# Autodesk Inventor assembly: Sorting Mechanism Assembly
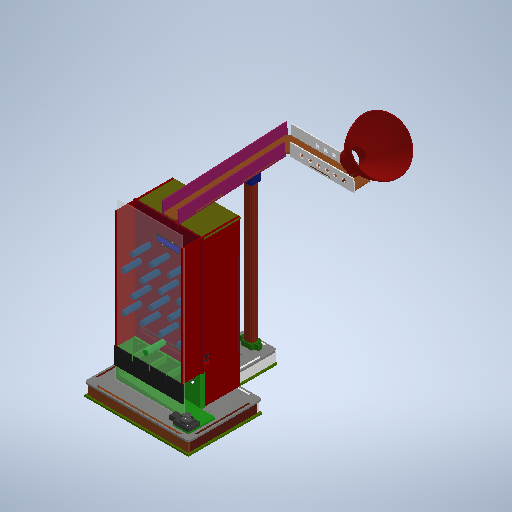
[picture p0: Inventor's stored thumbnail of the model, 512x512]
Saved by Autodesk Inventor 2025.4 (Build 294407000, 407)
## iProperties
Created: 2026-04-05
Part Number: Sorting Mechanism Assembly
Document SubType Name: Assembly
Designer: lenovo
Author: lenovo
## Documents named in this file (39)
- F:\ASU Engineering\Year.2 ( 25-26 )\Spring\Basics Of Mechatronics\Project\Mechanisms\Sorting Mechanism\Sorting Mechanism Assembly.iam
- F:\ASU Engineering\Year.2 ( 25-26 )\Spring\Basics Of Mechatronics\Project\Mechanisms\Sorting Mechanism\Base.ipt
- F:\ASU Engineering\Year.2 ( 25-26 )\Spring\Basics Of Mechatronics\Project\Mechanisms\Sorting Mechanism\Random Plate  ( Laser Cut ).ipt
- F:\ASU Engineering\Year.2 ( 25-26 )\Spring\Basics Of Mechatronics\Project\Mechanisms\Sorting Mechanism\Randomization Stick.ipt
- F:\ASU Engineering\Year.2 ( 25-26 )\Spring\Basics Of Mechatronics\Project\Mechanisms\Sorting Mechanism\Finishing Sheets .1  ( Right ).ipt
- F:\ASU Engineering\Year.2 ( 25-26 )\Spring\Basics Of Mechatronics\Project\Mechanisms\Sorting Mechanism\Rack ( Female Fixation ).ipt
- F:\ASU Engineering\Year.2 ( 25-26 )\Spring\Basics Of Mechatronics\Project\Mechanisms\Sorting Mechanism\Rack ( Male Fixation.ipt
- F:\ASU Engineering\Year.2 ( 25-26 )\Spring\Basics Of Mechatronics\Project\Mechanisms\Sorting Mechanism\Sorting Mechanism Base Fixation.ipt
- F:\ASU Engineering\Year.2 ( 25-26 )\Spring\Basics Of Mechatronics\Project\Mechanisms\Sorting Mechanism\Finishing Sheets .2  ( Upper ).ipt
- F:\ASU Engineering\Year.2 ( 25-26 )\Spring\Basics Of Mechatronics\Project\Mechanisms\Sorting Mechanism\Finishing Sheets .3  ( Back ).ipt
- F:\ASU Engineering\Year.2 ( 25-26 )\Spring\Basics Of Mechatronics\Project\Mechanisms\Sorting Mechanism\Finishing Sheets .4 ( Front )  Acrylic.ipt
- F:\ASU Engineering\Year.2 ( 25-26 )\Spring\Basics Of Mechatronics\Project\Mechanisms\Sorting Mechanism\Finishing Sheets .5 ( Buttom ).ipt
- F:\ASU Engineering\Year.2 ( 25-26 )\Spring\Basics Of Mechatronics\Project\Mechanisms\Sorting Mechanism\Joystick Shield.ipt
- F:\ASU Engineering\Year.2 ( 25-26 )\Spring\Basics Of Mechatronics\Project\Mechanisms\Sorting Mechanism\Base Leg V1.ipt
- F:\ASU Engineering\Year.2 ( 25-26 )\Spring\Basics Of Mechatronics\Project\Mechanisms\Sorting Mechanism\Base Leg V2.ipt
- F:\ASU Engineering\Year.2 ( 25-26 )\Spring\Basics Of Mechatronics\Project\Mechanisms\Sorting Mechanism\Movable Stick.ipt
- F:\ASU Engineering\Year.2 ( 25-26 )\Spring\Basics Of Mechatronics\Project\Mechanisms\Sorting Mechanism\Lower Path Fixation.ipt
- F:\ASU Engineering\Year.2 ( 25-26 )\Spring\Basics Of Mechatronics\Project\Mechanisms\Sorting Mechanism\Path Holder.ipt
- F:\ASU Engineering\Year.2 ( 25-26 )\Spring\Basics Of Mechatronics\Project\Mechanisms\Sorting Mechanism\Upper Path Fixation.ipt
- F:\ASU Engineering\Year.2 ( 25-26 )\Spring\Basics Of Mechatronics\Project\Mechanisms\Sorting Mechanism\Path.ipt
- F:\ASU Engineering\Year.2 ( 25-26 )\Spring\Basics Of Mechatronics\Project\Mechanisms\Sorting Mechanism\Path Side Wall.ipt
- F:\ASU Engineering\Year.2 ( 25-26 )\Spring\Basics Of Mechatronics\Project\Mechanisms\Sorting Mechanism\Path Back End.ipt
- F:\ASU Engineering\Year.2 ( 25-26 )\Spring\Basics Of Mechatronics\Project\Mechanisms\Sorting Mechanism\Cone FV.ipt
- F:\ASU Engineering\Year.2 ( 25-26 )\Spring\Basics Of Mechatronics\Project\Mechanisms\Sorting Mechanism\Path Base Fixation .1.ipt
- F:\ASU Engineering\Year.2 ( 25-26 )\Spring\Basics Of Mechatronics\Project\Mechanisms\Sorting Mechanism\Path Base Fixation .2.ipt
- F:\ASU Engineering\Year.2 ( 25-26 )\Spring\Basics Of Mechatronics\Project\Mechanisms\Sorting Mechanism\Sensors Shield.ipt
- F:\ASU Engineering\Year.2 ( 25-26 )\Spring\Basics Of Mechatronics\Project\Mechanisms\Sorting Mechanism\DC Gear Motor Single Shaft\DC Gear Motor Single Shaft\DC Gear Motor Single Shaft.ipt
- F:\ASU Engineering\Year.2 ( 25-26 )\Spring\Basics Of Mechatronics\Project\Mechanisms\Sorting Mechanism\IR Sensor\IR Sensor\IR Sensor.ipt
- F:\ASU Engineering\Year.2 ( 25-26 )\Spring\Basics Of Mechatronics\Project\Mechanisms\Sorting Mechanism\Limit_Switch\Limit_Switch\Limit_Switch.ipt
- F:\ASU Engineering\Year.2 ( 25-26 )\Spring\Basics Of Mechatronics\Project\Mechanisms\Sorting Mechanism\Joystick\Joystick\Joystick.ipt
- F:\ASU Engineering\Year.2 ( 25-26 )\Spring\Basics Of Mechatronics\Project\Mechanisms\Sorting Mechanism\Base Leg V2 Slotted.ipt
- F:\ASU Engineering\Year.2 ( 25-26 )\Spring\Basics Of Mechatronics\Project\Mechanisms\Sorting Mechanism\DC Motor Fixing Wall.ipt
- F:\ASU Engineering\Year.2 ( 25-26 )\Spring\Basics Of Mechatronics\Project\Mechanisms\Sorting Mechanism\Geared Motor Transmission.ipt
- F:\ASU Engineering\Year.2 ( 25-26 )\Spring\Basics Of Mechatronics\Project\Mechanisms\Sorting Mechanism\Pinion Gear FV.ipt
- F:\ASU Engineering\Year.2 ( 25-26 )\Spring\Basics Of Mechatronics\Project\Mechanisms\Sorting Mechanism\Path Plate Connector.ipt
- F:\ASU Engineering\Year.2 ( 25-26 )\Spring\Basics Of Mechatronics\Project\Mechanisms\Sorting Mechanism\LCD-I2C_16X2\LCD-I2C_16X2\LCD-I2C_16X2.iam
- F:\ASU Engineering\Year.2 ( 25-26 )\Spring\Basics Of Mechatronics\Project\Mechanisms\Sorting Mechanism\Extension .1.ipt
- F:\ASU Engineering\Year.2 ( 25-26 )\Spring\Basics Of Mechatronics\Project\Mechanisms\Sorting Mechanism\Extension.2.ipt
- F:\ASU Engineering\Year.2 ( 25-26 )\Spring\Basics Of Mechatronics\Project\Mechanisms\Sorting Mechanism\Extension .3.ipt
## Components (63 placed, 38 different names)
1. Base:1 — Mate:1, Mate:3, Flush:1, Mate:34, Mate:37, Mate:48, Mate:49, Mate:50, Mate:62, Mate:63, Mate:64, Mate:127, Mate:128, Mate:129, Mate:130, Mate:131, Mate:132, Mate:133, Mate:134, Mate:135, Mate:136, Mate:137, Mate:138, Mate:139, Mate:140, Mate:147, Mate:153, Mate:167, Mate:168, Mate:169
2. Random Plate  ( Laser Cut ):1 — Mate:1, Mate:3, Flush:1, Mate:4, Mate:5, Mate:6, Mate:7, Mate:8, Mate:9, Mate:10, Mate:11, Mate:12, Mate:13, Mate:14, Mate:15, Mate:16, Mate:17, Mate:18, Mate:19, Mate:20, Mate:21, Mate:22, Mate:23, Mate:24, Mate:25, Mate:26, Mate:27, Mate:28, Mate:29, Mate:30, Mate:31, Mate:32, Mate:33, Mate:35, Mate:36, Mate:38, Mate:39, Mate:40, Mate:51, Mate:59, Mate:79, Mate:80, Mate:124, Mate:175, Mate:177, Mate:178, Mate:179
3. Randomization Stick:1 — Mate:4, Mate:18
4. Randomization Stick:2 — Mate:8, Mate:20
5. Randomization Stick:3 — Mate:5, Mate:19
6. Randomization Stick:4 — Mate:7, Mate:27
7. Randomization Stick:5 — Mate:6, Mate:28
8. Randomization Stick:6 — Mate:9, Mate:30
9. Randomization Stick:7 — Mate:10, Mate:29
10. Randomization Stick:8 — Mate:11, Mate:21
11. Randomization Stick:9 — Mate:12, Mate:22
12. Randomization Stick:10 — Mate:14, Mate:31
13. Randomization Stick:11 — Mate:13, Mate:23
14. Randomization Stick:12 — Mate:16, Mate:25
15. Randomization Stick:13 — Mate:17, Mate:26
16. Randomization Stick:14 — Mate:15, Mate:24
17. Finishing Sheets .1  ( Right ):1 — Mate:32, Mate:33, Mate:34, Mate:80, Mate:126
18. Finishing Sheets .1  ( Right ):2 — Mate:35, Mate:36, Mate:37, Mate:52, Mate:53, Mate:55, Mate:56, Mate:60, Mate:61, Mate:79
19. Rack ( Female Fixation ):1 — Mate:38, Mate:39, Mate:40, Mate:41, Mate:42, Mate:155, Mate:156, Mate:157, Mate:158, Mate:159, Mate:160
20. Rack ( Male Fixation:1 — Mate:41, Mate:42, Mate:81, Mate:82, Rotation/Translation:1
21. Sorting Mechanism Base Fixation:1 — Mate:48, Mate:49, Mate:50, Mate:65, Mate:66, Mate:68, Mate:71, Mate:72, Mate:73, Mate:74, Mate:75, Mate:76, Mate:77, Flush:59, Mate:96, Mate:97, Mate:98, Mate:113, Mate:114, Mate:115, Mate:116, Mate:117, Mate:118, Mate:120, Mate:121, Mate:164, Mate:165, Mate:166
22. Finishing Sheets .2  ( Upper ):1 — Mate:59, Mate:60, Mate:61
23. Finishing Sheets .3  ( Back ):1 — Mate:51, Mate:52, Mate:53, Mate:54
24. Finishing Sheets .4 ( Front )  Acrylic:1 — Mate:54, Mate:55, Mate:56, Flush:110, Mate:125
25. Finishing Sheets .5 ( Buttom ):1 — Mate:77, Mate:78, Flush:59
26. Joystick Shield:1 — Mate:62, Mate:63, Mate:64, Mate:154, Flush:113
27. Base Leg V1:1 — Mate:72, Mate:73, Mate:75
28. Base Leg V2:1 — Mate:65, Mate:66, Mate:68, Mate:78
29. Base Leg V1:2 — Mate:71, Mate:74, Mate:76
30. Movable Stick:1 — Mate:81, Mate:82, Mate:124
31. Lower Path Fixation:1 — Mate:83, Mate:84, Mate:85, Mate:86, Mate:87, Mate:88, Mate:89, Mate:90, Mate:91, Mate:92, Mate:93, Mate:94, Mate:95, Mate:96, Mate:97, Mate:98, Flush:60, Mate:102, Mate:119
32. Path Holder:1 — Mate:83, Mate:93, Mate:94
33. Upper Path Fixation:1 — Flush:60, Mate:99, Mate:100, Mate:101, Mate:103, Mate:104, Mate:144, Mate:145, Mate:146
34. Path Holder:2 — Mate:84, Mate:87, Mate:92, Mate:99, Mate:100
35. Path Holder:3 — Mate:85, Mate:89, Mate:95
36. Path Holder:4 — Mate:86, Mate:88, Mate:90, Mate:91
37. Path:1 — Mate:101, Mate:102, Mate:103, Mate:104, Mate:105, Flush:61, Mate:106, Mate:141, Mate:142, Mate:143, Mate:184, Mate:185, Mate:186, Mate:192, Mate:193, Mate:194, Mate:195, Mate:196, Mate:197
38. Path Side Wall:1 — Mate:105, Flush:61, Mate:106
39. Path Back End:1 — Mate:187, Mate:188, Mate:189, Mate:190, Mate:191
40. Cone FV:1 — Mate:189, Mate:191
41. Path Base Fixation .1:1 — Mate:116, Mate:117, Mate:118
42. Path Base Fixation .1:2 — Mate:113, Mate:114, Mate:115
43. Path Base Fixation .2:1 — Mate:119, Mate:120, Mate:121
44. Sensors Shield:1 — Flush:110, Mate:125, Mate:126
45. DC Gear Motor Single Shaft:1 — Mate:127, Mate:128, Mate:147, Mate:170, Mate:171
46. IR Sensor:1 — Mate:135, Mate:136, Mate:137
47. IR Sensor:2 — Mate:138, Mate:139, Mate:140
48. IR Sensor:3 — Mate:132, Mate:133, Mate:134
49. IR Sensor:4 — Mate:129, Mate:130, Mate:131
50. IR Sensor:5 — Mate:144, Mate:145, Mate:146
51. IR Sensor:6 — Mate:141, Mate:142, Mate:143
52. Limit_Switch:1 — Mate:158, Mate:159, Mate:160
53. Limit_Switch:2 — Mate:155, Mate:156, Mate:157
54. Joystick:1 — Mate:153, Mate:154, Flush:113
55. Base Leg V2 Slotted:1 — Mate:164, Mate:165, Mate:166
56. DC Motor Fixing Wall:1 — Mate:167, Mate:168, Mate:169
57. Geared Motor Transmission:1 — Mate:170, Mate:171, Mate:172, Mate:173, Mate:174
58. Pinion Gear FV:1 — Mate:172, Mate:173, Mate:174, Rotation/Translation:1
59. Path Plate Connector:1 — Mate:175
60. LCD-I2C_16X2:1 [sub-assembly] — Mate:177, Mate:178, Mate:179
61. Extension .1:1 — Mate:184, Mate:185, Mate:186, Mate:187, Mate:188, Mate:190, Mate:192
62. Extension.2:1 — Mate:193, Mate:194, Mate:195
63. Extension .3:1 — Mate:196, Mate:197
## Relationships (172: Mate 165, Flush 6, RelateRotateTranslate 1)
- Mate:1: Base:1 ↔ Random Plate  ( Laser Cut ):1
- Mate:3: Base:1 ↔ Random Plate  ( Laser Cut ):1
- Flush:1: Base:1 ↔ Random Plate  ( Laser Cut ):1
- Mate:4: Random Plate  ( Laser Cut ):1 ↔ Randomization Stick:1
- Mate:5: Random Plate  ( Laser Cut ):1 ↔ Randomization Stick:3
- Mate:6: Random Plate  ( Laser Cut ):1 ↔ Randomization Stick:5
- Mate:7: Random Plate  ( Laser Cut ):1 ↔ Randomization Stick:4
- Mate:8: Random Plate  ( Laser Cut ):1 ↔ Randomization Stick:2
- Mate:9: Random Plate  ( Laser Cut ):1 ↔ Randomization Stick:6
- Mate:10: Random Plate  ( Laser Cut ):1 ↔ Randomization Stick:7
- Mate:11: Random Plate  ( Laser Cut ):1 ↔ Randomization Stick:8
- Mate:12: Random Plate  ( Laser Cut ):1 ↔ Randomization Stick:9
- Mate:13: Random Plate  ( Laser Cut ):1 ↔ Randomization Stick:11
- Mate:14: Random Plate  ( Laser Cut ):1 ↔ Randomization Stick:10
- Mate:15: Random Plate  ( Laser Cut ):1 ↔ Randomization Stick:14
- Mate:16: Random Plate  ( Laser Cut ):1 ↔ Randomization Stick:12
- Mate:17: Random Plate  ( Laser Cut ):1 ↔ Randomization Stick:13
- Mate:18: Random Plate  ( Laser Cut ):1 ↔ Randomization Stick:1
- Mate:19: Random Plate  ( Laser Cut ):1 ↔ Randomization Stick:3
- Mate:20: Random Plate  ( Laser Cut ):1 ↔ Randomization Stick:2
- Mate:21: Random Plate  ( Laser Cut ):1 ↔ Randomization Stick:8
- Mate:22: Random Plate  ( Laser Cut ):1 ↔ Randomization Stick:9
- Mate:23: Random Plate  ( Laser Cut ):1 ↔ Randomization Stick:11
- Mate:24: Random Plate  ( Laser Cut ):1 ↔ Randomization Stick:14
- Mate:25: Random Plate  ( Laser Cut ):1 ↔ Randomization Stick:12
- Mate:26: Random Plate  ( Laser Cut ):1 ↔ Randomization Stick:13
- Mate:27: Random Plate  ( Laser Cut ):1 ↔ Randomization Stick:4
- Mate:28: Random Plate  ( Laser Cut ):1 ↔ Randomization Stick:5
- Mate:29: Random Plate  ( Laser Cut ):1 ↔ Randomization Stick:7
- Mate:30: Random Plate  ( Laser Cut ):1 ↔ Randomization Stick:6
- Mate:31: Random Plate  ( Laser Cut ):1 ↔ Randomization Stick:10
- Mate:32: Random Plate  ( Laser Cut ):1 ↔ Finishing Sheets .1  ( Right ):1
- Mate:33: Random Plate  ( Laser Cut ):1 ↔ Finishing Sheets .1  ( Right ):1
- Mate:34: Base:1 ↔ Finishing Sheets .1  ( Right ):1
- Mate:35: Random Plate  ( Laser Cut ):1 ↔ Finishing Sheets .1  ( Right ):2
- Mate:36: Random Plate  ( Laser Cut ):1 ↔ Finishing Sheets .1  ( Right ):2
- Mate:37: Base:1 ↔ Finishing Sheets .1  ( Right ):2
- Mate:38: Random Plate  ( Laser Cut ):1 ↔ Rack ( Female Fixation ):1
- Mate:39: Random Plate  ( Laser Cut ):1 ↔ Rack ( Female Fixation ):1
- Mate:40: Random Plate  ( Laser Cut ):1 ↔ Rack ( Female Fixation ):1
- Mate:41: Rack ( Female Fixation ):1 ↔ Rack ( Male Fixation:1
- Mate:42: Rack ( Female Fixation ):1 ↔ Rack ( Male Fixation:1
- Mate:48: Base:1 ↔ Sorting Mechanism Base Fixation:1
- Mate:49: Base:1 ↔ Sorting Mechanism Base Fixation:1
- Mate:50: Base:1 ↔ Sorting Mechanism Base Fixation:1
- Mate:51: Random Plate  ( Laser Cut ):1 ↔ Finishing Sheets .3  ( Back ):1
- Mate:52: Finishing Sheets .1  ( Right ):2 ↔ Finishing Sheets .3  ( Back ):1
- Mate:53: Finishing Sheets .1  ( Right ):2 ↔ Finishing Sheets .3  ( Back ):1
- Mate:54: Finishing Sheets .3  ( Back ):1 ↔ Finishing Sheets .4 ( Front )  Acrylic:1
- Mate:55: Finishing Sheets .1  ( Right ):2 ↔ Finishing Sheets .4 ( Front )  Acrylic:1
- Mate:56: Finishing Sheets .1  ( Right ):2 ↔ Finishing Sheets .4 ( Front )  Acrylic:1
- Mate:59: Random Plate  ( Laser Cut ):1 ↔ Finishing Sheets .2  ( Upper ):1
- Mate:60: Finishing Sheets .1  ( Right ):2 ↔ Finishing Sheets .2  ( Upper ):1
- Mate:61: Finishing Sheets .1  ( Right ):2 ↔ Finishing Sheets .2  ( Upper ):1
- Mate:62: Base:1 ↔ Joystick Shield:1
- Mate:63: Base:1 ↔ Joystick Shield:1
- Mate:64: Base:1 ↔ Joystick Shield:1
- Mate:65: Sorting Mechanism Base Fixation:1 ↔ Base Leg V2:1
- Mate:66: Sorting Mechanism Base Fixation:1 ↔ Base Leg V2:1
- Mate:68: Sorting Mechanism Base Fixation:1 ↔ Base Leg V2:1
- Mate:71: Sorting Mechanism Base Fixation:1 ↔ Base Leg V1:2
- Mate:72: Sorting Mechanism Base Fixation:1 ↔ Base Leg V1:1
- Mate:73: Sorting Mechanism Base Fixation:1 ↔ Base Leg V1:1
- Mate:74: Sorting Mechanism Base Fixation:1 ↔ Base Leg V1:2
- Mate:75: Sorting Mechanism Base Fixation:1 ↔ Base Leg V1:1
- Mate:76: Sorting Mechanism Base Fixation:1 ↔ Base Leg V1:2
- Mate:77: Sorting Mechanism Base Fixation:1 ↔ Finishing Sheets .5 ( Buttom ):1
- Mate:78: Finishing Sheets .5 ( Buttom ):1 ↔ Base Leg V2:1
- Flush:59: Sorting Mechanism Base Fixation:1 ↔ Finishing Sheets .5 ( Buttom ):1
- Mate:79: Random Plate  ( Laser Cut ):1 ↔ Finishing Sheets .1  ( Right ):2
- Mate:80: Random Plate  ( Laser Cut ):1 ↔ Finishing Sheets .1  ( Right ):1
- Mate:81: Rack ( Male Fixation:1 ↔ Movable Stick:1
- Mate:82: Rack ( Male Fixation:1 ↔ Movable Stick:1
- Mate:83: Lower Path Fixation:1 ↔ Path Holder:1
- Mate:84: Lower Path Fixation:1 ↔ Path Holder:2
- Mate:85: Lower Path Fixation:1 ↔ Path Holder:3
- Mate:86: Lower Path Fixation:1 ↔ Path Holder:4
- Mate:87: Lower Path Fixation:1 ↔ Path Holder:2
- Mate:88: Lower Path Fixation:1 ↔ Path Holder:4
- Mate:89: Lower Path Fixation:1 ↔ Path Holder:3
- Mate:90: Lower Path Fixation:1 ↔ Path Holder:4
- Mate:91: Lower Path Fixation:1 ↔ Path Holder:4
- Mate:92: Lower Path Fixation:1 ↔ Path Holder:2
- Mate:93: Lower Path Fixation:1 ↔ Path Holder:1
- Mate:94: Lower Path Fixation:1 ↔ Path Holder:1
- Mate:95: Lower Path Fixation:1 ↔ Path Holder:3
- Mate:96: Sorting Mechanism Base Fixation:1 ↔ Lower Path Fixation:1
- Mate:97: Sorting Mechanism Base Fixation:1 ↔ Lower Path Fixation:1
- Mate:98: Sorting Mechanism Base Fixation:1 ↔ Lower Path Fixation:1
- Flush:60: Lower Path Fixation:1 ↔ Upper Path Fixation:1
- Mate:99: Upper Path Fixation:1 ↔ Path Holder:2
- Mate:100: Upper Path Fixation:1 ↔ Path Holder:2
- Mate:101: Upper Path Fixation:1 ↔ Path:1
- Mate:102: Lower Path Fixation:1 ↔ Path:1
- Mate:103: Upper Path Fixation:1 ↔ Path:1
- Mate:104: Upper Path Fixation:1 ↔ Path:1
- Mate:105: Path:1 ↔ Path Side Wall:1
- Flush:61: Path:1 ↔ Path Side Wall:1
- Mate:106: Path:1 ↔ Path Side Wall:1
- Mate:113: Sorting Mechanism Base Fixation:1 ↔ Path Base Fixation .1:2
- Mate:114: Sorting Mechanism Base Fixation:1 ↔ Path Base Fixation .1:2
- Mate:115: Sorting Mechanism Base Fixation:1 ↔ Path Base Fixation .1:2
- Mate:116: Sorting Mechanism Base Fixation:1 ↔ Path Base Fixation .1:1
- Mate:117: Sorting Mechanism Base Fixation:1 ↔ Path Base Fixation .1:1
- Mate:118: Sorting Mechanism Base Fixation:1 ↔ Path Base Fixation .1:1
- Mate:119: Lower Path Fixation:1 ↔ Path Base Fixation .2:1
- Mate:120: Sorting Mechanism Base Fixation:1 ↔ Path Base Fixation .2:1
- Mate:121: Sorting Mechanism Base Fixation:1 ↔ Path Base Fixation .2:1
- Mate:124: Random Plate  ( Laser Cut ):1 ↔ Movable Stick:1
- Flush:110: Finishing Sheets .4 ( Front )  Acrylic:1 ↔ Sensors Shield:1
- Mate:125: Finishing Sheets .4 ( Front )  Acrylic:1 ↔ Sensors Shield:1
- Mate:126: Finishing Sheets .1  ( Right ):1 ↔ Sensors Shield:1
- Mate:127 (3 mm): Base:1 ↔ DC Gear Motor Single Shaft:1
- Mate:128: Base:1 ↔ DC Gear Motor Single Shaft:1
- Mate:129: Base:1 ↔ IR Sensor:4
- Mate:130: Base:1 ↔ IR Sensor:4
- Mate:131: Base:1 ↔ IR Sensor:4
- Mate:132: Base:1 ↔ IR Sensor:3
- Mate:133: Base:1 ↔ IR Sensor:3
- Mate:134 (23 mm): Base:1 ↔ IR Sensor:3
- Mate:135: Base:1 ↔ IR Sensor:1
- Mate:136: Base:1 ↔ IR Sensor:1
- Mate:137: Base:1 ↔ IR Sensor:1
- Mate:138: Base:1 ↔ IR Sensor:2
- Mate:139: Base:1 ↔ IR Sensor:2
- Mate:140: Base:1 ↔ IR Sensor:2
- Mate:141: Path:1 ↔ IR Sensor:6
- Mate:142: Path:1 ↔ IR Sensor:6
- Mate:143: Path:1 ↔ IR Sensor:6
- Mate:144: Upper Path Fixation:1 ↔ IR Sensor:5
- Mate:145: Upper Path Fixation:1 ↔ IR Sensor:5
- Mate:146: Upper Path Fixation:1 ↔ IR Sensor:5
- Mate:147: Base:1 ↔ DC Gear Motor Single Shaft:1
- Mate:153: Base:1 ↔ Joystick:1
- Mate:154: Joystick Shield:1 ↔ Joystick:1
- Flush:113: Joystick Shield:1 ↔ Joystick:1
- Mate:155: Rack ( Female Fixation ):1 ↔ Limit_Switch:2
- Mate:156: Rack ( Female Fixation ):1 ↔ Limit_Switch:2
- Mate:157: Rack ( Female Fixation ):1 ↔ Limit_Switch:2
- Mate:158: Rack ( Female Fixation ):1 ↔ Limit_Switch:1
- Mate:159: Rack ( Female Fixation ):1 ↔ Limit_Switch:1
- Mate:160: Rack ( Female Fixation ):1 ↔ Limit_Switch:1
- Mate:164: Sorting Mechanism Base Fixation:1 ↔ Base Leg V2 Slotted:1
- Mate:165: Sorting Mechanism Base Fixation:1 ↔ Base Leg V2 Slotted:1
- Mate:166: Sorting Mechanism Base Fixation:1 ↔ Base Leg V2 Slotted:1
- Mate:167: Base:1 ↔ DC Motor Fixing Wall:1
- Mate:168: Base:1 ↔ DC Motor Fixing Wall:1
- Mate:169: Base:1 ↔ DC Motor Fixing Wall:1
- Mate:170: DC Gear Motor Single Shaft:1 ↔ Geared Motor Transmission:1
- Mate:171 (0.7 mm): DC Gear Motor Single Shaft:1 ↔ Geared Motor Transmission:1
- Mate:172: Geared Motor Transmission:1 ↔ Pinion Gear FV:1
- Mate:173: Geared Motor Transmission:1 ↔ Pinion Gear FV:1
- Mate:174: Geared Motor Transmission:1 ↔ Pinion Gear FV:1
- Rotation/Translation:1 [RelateRotateTranslate] (-70 mm): Rack ( Male Fixation:1 ↔ Pinion Gear FV:1
- Mate:175: Random Plate  ( Laser Cut ):1 ↔ Path Plate Connector:1
- Mate:177: Random Plate  ( Laser Cut ):1 ↔ LCD-I2C_16X2:1
- Mate:178: Random Plate  ( Laser Cut ):1 ↔ LCD-I2C_16X2:1
- Mate:179: Random Plate  ( Laser Cut ):1 ↔ LCD-I2C_16X2:1
- Mate:184: Path:1 ↔ Extension .1:1
- Mate:185: Path:1 ↔ Extension .1:1
- Mate:186: Path:1 ↔ Extension .1:1
- Mate:187: Path Back End:1 ↔ Extension .1:1
- Mate:188: Path Back End:1 ↔ Extension .1:1
- Mate:189: Path Back End:1 ↔ Cone FV:1
- Mate:190: Path Back End:1 ↔ Extension .1:1
- Mate:191: Path Back End:1 ↔ Cone FV:1
- Mate:192: Path:1 ↔ Extension .1:1
- Mate:193: Path:1 ↔ Extension.2:1
- Mate:194: Path:1 ↔ Extension.2:1
- Mate:195: Path:1 ↔ Extension.2:1
- Mate:196: Path:1 ↔ Extension .3:1
- Mate:197: Path:1 ↔ Extension .3:1
